# Autodesk Inventor assembly: speedometr2
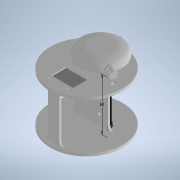
[picture p0: Inventor's stored thumbnail of the model, 180x180]
Saved by Autodesk Inventor 2022 (Build 260153000, 153)
## iProperties
Created: 2025-06-18
Part Number: speedometr2
Document SubType Name: Assembly
Designer: korsh624
Author: korsh624
## Documents named in this file (5)
- C:\git\izhplaneta5\speedmetr\models\speedometr2.iam
- C:\git\izhplaneta5\speedmetr\models\PX4 Neo M8N GPS.ipt
- C:\git\izhplaneta5\speedmetr\models\I2C OLED 128×64 Display Module.ipt
- C:\git\izhplaneta5\speedmetr\models\top.ipt
- C:\git\izhplaneta5\speedmetr\models\MEGA 2560 PRO.ipt
## Components (4 placed, 4 different names)
1. PX4 Neo M8N GPS:1 — Совмещение:1
2. I2C OLED 128×64 Display Module:1 — Совмещение:2, Совмещение:3, Совмещение:4
3. top:1 — Совмещение:1, Совмещение:2, Совмещение:3, Совмещение:4, Совмещение:5
4. MEGA 2560 PRO:1 — Совмещение:5
## Relationships (5: Mate 5)
- Совмещение:1 [Mate]: PX4 Neo M8N GPS:1 ↔ top:1
- Совмещение:2 [Mate]: I2C OLED 128×64 Display Module:1 ↔ top:1
- Совмещение:3 [Mate]: I2C OLED 128×64 Display Module:1 ↔ top:1
- Совмещение:4 [Mate]: I2C OLED 128×64 Display Module:1 ↔ top:1
- Совмещение:5 [Mate] (2 mm): top:1 ↔ MEGA 2560 PRO:1
